# Autodesk Inventor assembly: Pneumatics_Clippard_AVT-32-32
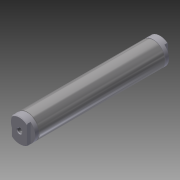
[picture p0: Inventor's stored thumbnail of the model, 180x180]
Saved by Autodesk Inventor 2014 SP1 (Build 180222100, 222)
## iProperties
Category: Pneumatics
Created: 2007-11-13
Part Number: Pneumatics_Clippard_AVT-32-32
Document SubType Name: Assembly
Catalog Web Link: http://www.clippard.com/store/display_details.asp?sku=AVT-32-16
Description: Accumulator
Vendor: Clippard
Mass: 1023.26 g
Surface Area: 1002.07 cm^2
Volume: 163.83 cm^3
Density: 6.24587 g/cm^3
Project: FIRST
Title: Accumulator
Author: Autodesk, Inc.
## Documents named in this file (3)
- C:\Users\Arpan\Documents\GitHub\2014buildCAD\big air tank\Pneumatics_Clippard_AVT-32-32.iam
- C:\Users\Arpan\Documents\GitHub\2014buildCAD\big air tank\AVT-32-32_End Cap.ipt
- C:\Users\Arpan\Documents\GitHub\2014buildCAD\big air tank\AVT-32-32_Body Tube.ipt
## Components (3 placed, 2 different names)
1. AVT-32-32_Body Tube:1 — Insert:1, Insert:2, Angle:1, Angle:2
2. AVT-32-32_End Cap:1 — Insert:1, Angle:1
3. AVT-32-32_End Cap:2 — Insert:2, Angle:2
## Relationships (4: Insert 2, Angle 2)
- Insert:1: AVT-32-32_Body Tube:1 ↔ AVT-32-32_End Cap:1
- Insert:2: AVT-32-32_Body Tube:1 ↔ AVT-32-32_End Cap:2
- Angle:1 (0 deg): AVT-32-32_Body Tube:1 ↔ AVT-32-32_End Cap:1
- Angle:2 (0 deg): AVT-32-32_Body Tube:1 ↔ AVT-32-32_End Cap:2
